# Autodesk Inventor assembly: omni_harf_frame
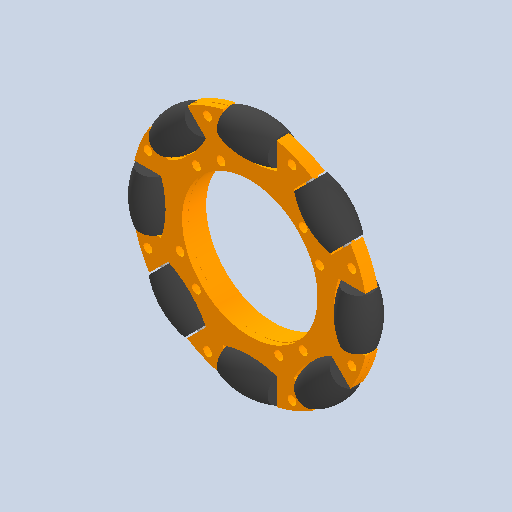
[picture p0: Inventor's stored thumbnail of the model, 512x512]
Saved by Autodesk Inventor 2024.1 (Build 281209000, 209)
## iProperties
Created: 2024-11-26
Part Number: omni_harf_frame
Document SubType Name: Assembly
Designer: hibik
Author: hibik
## Documents named in this file (4)
- C:\Users\hibik\Documents\Robomech\RESCUE\ORCA\hard\omni_wheel\omni_harf_frame.iam
- C:\Users\hibik\Documents\Robomech\RESCUE\ORCA\hard\omni_wheel\wheel_body_back.ipt
- C:\Users\hibik\Documents\Robomech\RESCUE\ORCA\hard\omni_wheel\roller.ipt
- C:\Users\hibik\Documents\Robomech\RESCUE\ORCA\hard\omni_wheel\wheel_body_front.ipt
## Components (10 placed, 3 different names)
1. wheel_body_back:1 — 正接:1, 正接:2, メイト:1, 正接:3, 正接:4, メイト:2, 正接:5, 正接:6, メイト:3, 正接:7, 正接:8, メイト:4, 正接:9, 正接:10, メイト:5, 正接:11, 正接:12, メイト:6, 正接:13, 正接:14, メイト:7, 正接:15, 正接:16, メイト:8, 挿入:1, 挿入:2
2. roller:1 — 正接:1, 正接:2, メイト:1
3. roller:2 — 正接:3, 正接:4, メイト:2
4. roller:3 — 正接:5, 正接:6, メイト:3
5. roller:4 — 正接:7, 正接:8, メイト:4
6. roller:5 — 正接:9, 正接:10, メイト:5
7. roller:6 — 正接:11, 正接:12, メイト:6
8. roller:7 — 正接:13, 正接:14, メイト:7
9. roller:8 — 正接:15, 正接:16, メイト:8
10. wheel_body_front:1 — 挿入:1, 挿入:2
## Relationships (26: Tangent 16, Mate 8, Insert 2)
- 正接:1 [Tangent]: wheel_body_back:1 ↔ roller:1
- 正接:2 [Tangent]: wheel_body_back:1 ↔ roller:1
- メイト:1 [Mate] (0.5 mm): wheel_body_back:1 ↔ roller:1
- 正接:3 [Tangent]: wheel_body_back:1 ↔ roller:2
- 正接:4 [Tangent]: wheel_body_back:1 ↔ roller:2
- メイト:2 [Mate] (0.5 mm): wheel_body_back:1 ↔ roller:2
- 正接:5 [Tangent]: wheel_body_back:1 ↔ roller:3
- 正接:6 [Tangent]: wheel_body_back:1 ↔ roller:3
- メイト:3 [Mate] (0.5 mm): wheel_body_back:1 ↔ roller:3
- 正接:7 [Tangent]: wheel_body_back:1 ↔ roller:4
- 正接:8 [Tangent]: wheel_body_back:1 ↔ roller:4
- メイト:4 [Mate] (0.5 mm): wheel_body_back:1 ↔ roller:4
- 正接:9 [Tangent]: wheel_body_back:1 ↔ roller:5
- 正接:10 [Tangent]: wheel_body_back:1 ↔ roller:5
- メイト:5 [Mate] (0.5 mm): wheel_body_back:1 ↔ roller:5
- 正接:11 [Tangent]: wheel_body_back:1 ↔ roller:6
- 正接:12 [Tangent]: wheel_body_back:1 ↔ roller:6
- メイト:6 [Mate] (0.5 mm): wheel_body_back:1 ↔ roller:6
- 正接:13 [Tangent]: wheel_body_back:1 ↔ roller:7
- 正接:14 [Tangent]: wheel_body_back:1 ↔ roller:7
- メイト:7 [Mate] (0.5 mm): wheel_body_back:1 ↔ roller:7
- 正接:15 [Tangent]: wheel_body_back:1 ↔ roller:8
- 正接:16 [Tangent]: wheel_body_back:1 ↔ roller:8
- メイト:8 [Mate] (0.5 mm): wheel_body_back:1 ↔ roller:8
- 挿入:1 [Insert]: wheel_body_back:1 ↔ wheel_body_front:1
- 挿入:2 [Insert]: wheel_body_back:1 ↔ wheel_body_front:1
